# Autodesk Inventor assembly: BackLowerLink
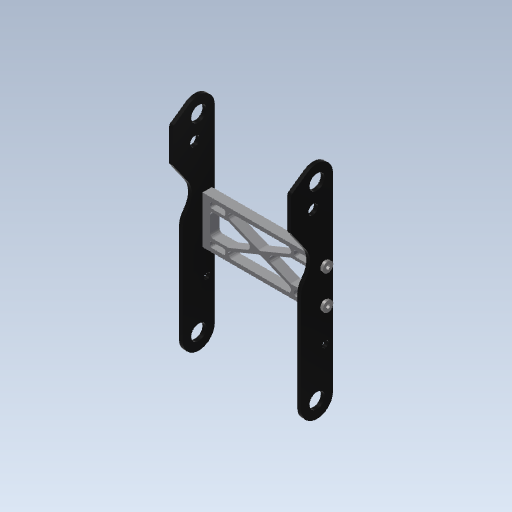
[picture p0: Inventor's stored thumbnail of the model, 512x512]
Saved by Autodesk Inventor 2020 (Build 240168000, 168)
## iProperties
Created: 2016-08-23
Part Number: BackLowerLink
Material: 一般
Document SubType Name: Assembly
Designer: hiro
Mass: 27.0677 g
Surface Area: 148.123 cm^2
Volume: 12.1706 cm^3
Density: 2.22402 g/cm^3
Author: hiro
## Documents named in this file (4)
- C:\Users\MasatoKubotera\Documents\Inventor\OpenPlatform_ver3_0 - sustaina_ver1_1_171\LowerBody\Link\BackLowerLink.iam
- C:\Users\MasatoKubotera\Documents\Inventor\OpenPlatform_ver3_0 - sustaina_ver1_1_171\ReadyMade\Screw\M3-6.ipt
- C:\Users\MasatoKubotera\Documents\Inventor\OpenPlatform_ver3_0 - sustaina_ver1_1_171\LowerBody\Link\BackLink_frame.ipt
- C:\Users\MasatoKubotera\Documents\Inventor\OpenPlatform_ver3_0 - sustaina_ver1_1_171\LowerBody\Link\BackLink_diagonal.ipt
## Components (7 placed, 3 different names)
1. BackLink_diagonal_:1 — 挿入:5, 挿入:6, 挿入:7, 挿入:8, メイト:1, メイト:2, フラッシュ:1
2. BackLink_frame:1 — 挿入:1, 挿入:2, 挿入:5, 挿入:6
3. BackLink_frame:2 — 挿入:3, 挿入:4, 挿入:7, 挿入:8
4. M3-6:1 — 挿入:2
5. M3-6:2 — 挿入:1
6. M3-6:3 — 挿入:4
7. M3-6:4 — 挿入:3
## Relationships (11: Insert 8, Mate 2, Flush 1)
- 挿入:1 [Insert]: BackLink_frame:1 ↔ M3-6:2
- 挿入:2 [Insert]: BackLink_frame:1 ↔ M3-6:1
- 挿入:3 [Insert]: BackLink_frame:2 ↔ M3-6:4
- 挿入:4 [Insert]: BackLink_frame:2 ↔ M3-6:3
- 挿入:5 [Insert]: BackLink_diagonal_:1 ↔ BackLink_frame:1
- 挿入:6 [Insert]: BackLink_diagonal_:1 ↔ BackLink_frame:1
- 挿入:7 [Insert]: BackLink_diagonal_:1 ↔ BackLink_frame:2
- 挿入:8 [Insert]: BackLink_diagonal_:1 ↔ BackLink_frame:2
- メイト:1 [Mate]: BackLink_diagonal_:1
- メイト:2 [Mate]: BackLink_diagonal_:1
- フラッシュ:1 [Flush]: BackLink_diagonal_:1
